# Autodesk Inventor assembly: ShelfLabel_Bütün
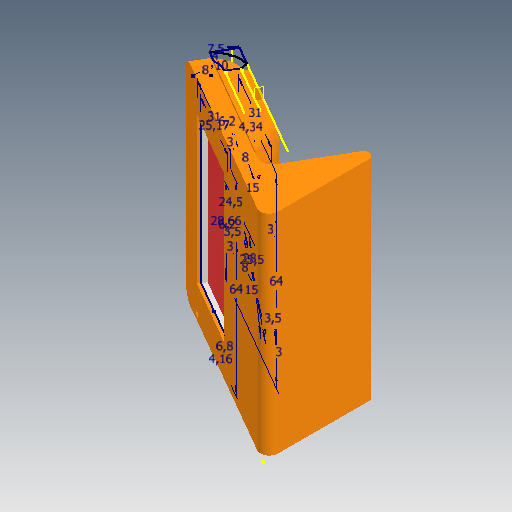
[picture p0: Inventor's stored thumbnail of the model, 512x512]
Saved by Autodesk Inventor 2020.3 (Build 243373000, 373)
## iProperties
Created: 2021-08-20
Part Number: ShelfLabel_Bütün
Document SubType Name: Assembly
Designer: Yusuf
Mass: 60.0499 g
Surface Area: 306.427 cm^2
Volume: 60.0499 cm^3
Density: 1 g/cm^3
Author: Yusuf
## Documents named in this file (5)
- C:\Users\Yusuf\Desktop\BordaAcademy_BoxDesign\ShelfLabel\ShelfLabel_Bütün.iam
- C:\Users\Yusuf\Desktop\BordaAcademy_BoxDesign\ShelfLabel\CR2450.ipt
- C:\Users\Yusuf\Desktop\BordaAcademy_BoxDesign\ShelfLabel\ShelfLabel.ipt
- C:\Users\Yusuf\Desktop\BordaAcademy_BoxDesign\ShelfLabel\ShelfLabelStand.ipt
- C:\Users\Yusuf\Desktop\BordaAcademy_BoxDesign\ShelfLabel\ShelfLabel-Kapak.ipt
## Components (5 placed, 4 different names)
1. CR2450:1 — Mate:5, Mate:7, Mate:10, Mate:12
2. ShelfLabel:1 — Mate:3, Mate:4, Mate:5, Mate:6, Mate:7, Mate:8, Mate:11
3. ShelfLabelStand:1 — Mate:3, Mate:4, Angle:1, Mate:11
4. CR2450:2 — Mate:6, Mate:8, Mate:9
5. ShelfLabel-Kapak:1 — Mate:9, Mate:10, Angle:1, Mate:12
## Relationships (11: Mate 10, Angle 1)
- Mate:3: ShelfLabel:1 ↔ ShelfLabelStand:1
- Mate:4: ShelfLabel:1 ↔ ShelfLabelStand:1
- Mate:5: CR2450:1 ↔ ShelfLabel:1
- Mate:6: ShelfLabel:1 ↔ CR2450:2
- Mate:7: CR2450:1 ↔ ShelfLabel:1
- Mate:8: ShelfLabel:1 ↔ CR2450:2
- Mate:9: CR2450:2 ↔ ShelfLabel-Kapak:1
- Mate:10: CR2450:1 ↔ ShelfLabel-Kapak:1
- Angle:1 (180 deg): ShelfLabelStand:1 ↔ ShelfLabel-Kapak:1
- Mate:11: ShelfLabel:1 ↔ ShelfLabelStand:1
- Mate:12: CR2450:1 ↔ ShelfLabel-Kapak:1
